# Autodesk Inventor assembly: R07-100-RNEA
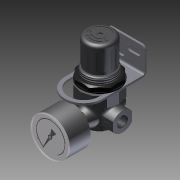
[picture p0: Inventor's stored thumbnail of the model, 180x180]
Saved by Autodesk Inventor 2015 SP1 (Build 190203100, 203)
## iProperties
Category: Pneumatics
Company: Autodesk Inc.
Created: 2014-12-16
Part Number: R07-100-RNEA
Document SubType Name: Assembly
Designer: Autodesk Inc.
Catalog Web Link: http://www.norgren.com/document_resources/EN/8.300.200.PDF
Vendor: Norgren
Description: Main Regulator (assembled)
Author: Autodesk Inc.
## Documents named in this file (5)
- D:\Data Folder\FIRST 2015\KOP_FRC\FirstChoice\Pneumatics_Norgren_R07-100-RNEA.iam
- D:\Data Folder\FIRST 2015\KOP_FRC\FirstChoice\Parts\Pneumatics_Norgren_R07-100-RNEA.ipt
- D:\Data Folder\FIRST 2015\KOP_FRC\FirstChoice\Parts\Pneumatics_Norgren_18-025-003_Bracket.ipt
- D:\Data Folder\FIRST 2015\KOP_FRC\FirstChoice\Parts\Pneumatics_Norgren_18-025-003_Panel Nut.ipt
- D:\Data Folder\FIRST 2015\KOP_FRC\FirstChoice\Parts\Pneumatics_Norgren_18-013-212.iam
## Components (4 placed, 4 different names)
1. Pneumatics_Norgren_R07-100-RNEA:1 — Mate:1, Mate:2, Mate:3, Insert:1
2. Pneumatics_Norgren_18-025-003_Bracket:1 — Mate:1, Mate:2, Mate:4
3. Pneumatics_Norgren_18-025-003_Panel Nut:1 — Mate:3, Mate:4
4. Pneumatics_Norgren_18-013-212:1 [sub-assembly] — Insert:1
## Relationships (5: Mate 4, Insert 1)
- Mate:1: Pneumatics_Norgren_R07-100-RNEA:1 ↔ Pneumatics_Norgren_18-025-003_Bracket:1
- Mate:2: Pneumatics_Norgren_R07-100-RNEA:1 ↔ Pneumatics_Norgren_18-025-003_Bracket:1
- Mate:3: Pneumatics_Norgren_R07-100-RNEA:1 ↔ Pneumatics_Norgren_18-025-003_Panel Nut:1
- Mate:4: Pneumatics_Norgren_18-025-003_Bracket:1 ↔ Pneumatics_Norgren_18-025-003_Panel Nut:1
- Insert:1: Pneumatics_Norgren_R07-100-RNEA:1 ↔ Pneumatics_Norgren_18-013-212:1
